# Autodesk Inventor assembly: PS20031
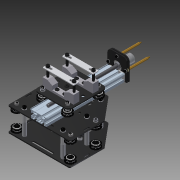
[picture p0: Inventor's stored thumbnail of the model, 180x180]
Saved by Autodesk Inventor 2014 (Build 180170000, 170)
## iProperties
Created: 2013-11-25
Part Number: PS20031
Document SubType Name: Assembly
Designer: Edward
Author: Edward
## Documents named in this file (8)
- C:\Users\Edward\Documents\GitHub\Shapeoko_2\Autodesk_Inventor_Project\PS20031.iam
- C:\Users\Edward\Documents\GitHub\Shapeoko_2\Autodesk_Inventor_Project\PS20022.iam
- C:\Users\Edward\Documents\GitHub\Shapeoko_2\Autodesk_Inventor_Project\PS20030.iam
- C:\Users\Edward\Documents\GitHub\Shapeoko_2\Autodesk_Inventor_Project\25312-20.ipt
- C:\Users\Edward\Documents\GitHub\Shapeoko_2\Autodesk_Inventor_Project\PS20006.ipt
- C:\Users\Edward\Documents\GitHub\Shapeoko_2\Autodesk_Inventor_Project\25287-02.ipt
- C:\Users\Edward\Documents\GitHub\Shapeoko_2\Autodesk_Inventor_Project\PS20002.ipt
- C:\Users\Edward\Documents\GitHub\Shapeoko_2\Autodesk_Inventor_Project\25284-02.ipt
## Components (38 placed, 7 different names)
1. PS20022:1 [sub-assembly] — Mate:1, Mate:2, Mate:3, Mate:4, Mate:5, Mate:6, Insert:6, Insert:7, Insert:37, Insert:38, Insert:39, Insert:40, Insert:41
2. PS20030:1 [sub-assembly] — Mate:1, Mate:2, Mate:3, Mate:4, Mate:5, Mate:6, Insert:4, Insert:5, Insert:24, Insert:28, Insert:29, Insert:30, Insert:31, Insert:32, Insert:33, Insert:34, Insert:35, Insert:36
3. 25312-20:1 — Insert:5
4. PS20006:1
5. 25287-02:1 — Insert:4
6. PS20002:1 — Insert:6
7. 25284-02:1
8. 25287-02:2 — Insert:7
9. 25312-20:2 — Insert:32
10. PS20002:2
11. 25284-02:2
12. 25287-02:4 — Insert:37
13. PS20006:3
14. 25287-02:5 — Insert:24
15. 25312-20:4 — Insert:33
16. PS20006:4
17. 25287-02:7 — Insert:29
18. PS20002:4
19. 25284-02:4
20. 25287-02:8 — Insert:40
21. 25312-20:5 — Insert:34
22. PS20006:5
23. 25287-02:9 — Insert:28
24. PS20002:5
25. 25284-02:5
26. 25287-02:10 — Insert:41
27. 25312-20:6 — Insert:35
28. PS20006:6
29. 25287-02:11 — Insert:30
30. PS20002:6
31. 25284-02:6
32. 25287-02:12 — Insert:39
33. 25312-20:7 — Insert:36
34. PS20006:7
35. 25287-02:13 — Insert:31
36. PS20002:7
37. 25284-02:7
38. 25287-02:14 — Insert:38
## Relationships (43: Insert 37, Mate 6)
- [Insert]: PS20006:1 ↔ 25287-02:1
- [Insert]: 25312-20:1 ↔ PS20002:1
- [Insert]: 25284-02:1 ↔ 25287-02:2
- Mate:1: PS20022:1 ↔ PS20030:1
- Mate:2: PS20022:1 ↔ PS20030:1
- Mate:3: PS20022:1 ↔ PS20030:1
- Mate:4: PS20022:1 ↔ PS20030:1
- Mate:5: PS20022:1 ↔ PS20030:1
- Mate:6: PS20022:1 ↔ PS20030:1
- Insert:4: PS20030:1 ↔ 25287-02:1
- Insert:5: PS20030:1 ↔ 25312-20:1
- Insert:6: PS20022:1 ↔ PS20002:1
- Insert:7: PS20022:1 ↔ 25287-02:2
- [Insert]: 25312-20:2 ↔ PS20002:2
- [Insert]: 25284-02:2 ↔ 25287-02:4
- [Insert]: PS20006:3 ↔ 25287-02:5
- [Insert]: PS20006:4 ↔ 25287-02:7
- [Insert]: 25312-20:4 ↔ PS20002:4
- [Insert]: 25284-02:4 ↔ 25287-02:8
- [Insert]: PS20006:5 ↔ 25287-02:9
- [Insert]: 25312-20:5 ↔ PS20002:5
- [Insert]: 25284-02:5 ↔ 25287-02:10
- [Insert]: PS20006:6 ↔ 25287-02:11
- [Insert]: 25312-20:6 ↔ PS20002:6
- [Insert]: 25284-02:6 ↔ 25287-02:12
- Insert:24: PS20030:1 ↔ 25287-02:5
- [Insert]: PS20006:7 ↔ 25287-02:13
- [Insert]: 25312-20:7 ↔ PS20002:7
- [Insert]: 25284-02:7 ↔ 25287-02:14
- Insert:28: PS20030:1 ↔ 25287-02:9
- Insert:29: PS20030:1 ↔ 25287-02:7
- Insert:30: PS20030:1 ↔ 25287-02:11
- Insert:31: PS20030:1 ↔ 25287-02:13
- Insert:32: PS20030:1 ↔ 25312-20:2
- Insert:33: PS20030:1 ↔ 25312-20:4
- Insert:34: PS20030:1 ↔ 25312-20:5
- Insert:35: PS20030:1 ↔ 25312-20:6
- Insert:36: PS20030:1 ↔ 25312-20:7
- Insert:37: PS20022:1 ↔ 25287-02:4
- Insert:38: PS20022:1 ↔ 25287-02:14
- Insert:39: PS20022:1 ↔ 25287-02:12
- Insert:40: PS20022:1 ↔ 25287-02:8
- Insert:41: PS20022:1 ↔ 25287-02:10
## Named parameters: d394_d372_d364 = 0 mm, d13_d394_d372_d364 = 0 mm, d14_d361 = 0 mm, d18_d359 = 0 mm, d19_d394_d372_d364 = 0 mm, d20_d361 = 0 mm, d21_d359 = 0 mm, d22_d394_d372_d364 = 0 mm, d23_d361 = 0 mm, d24_d359 = 0 mm, d25_d394_d372_d364 = 0 mm, d26_d361 = 0 mm, d27_d359 = 0 mm, d30_d394_d372_d364 = 0 mm, d31_d361 = 0 mm, d32_d359 = 0 mm
